# Autodesk Inventor assembly: IFI_FlyWheelAssembly_Jan21
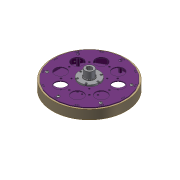
[picture p0: Inventor's stored thumbnail of the model, 180x180]
Saved by Autodesk Inventor 2012 (Build 160160000, 160)
## iProperties
Created: 2012-01-22
Part Number: IFI_FlyWheelAssembly_Jan21
Document SubType Name: Assembly
Designer: JesseK
Mass: 1834.43 g
Surface Area: 3040.14 cm^2
Volume: 862.441 cm^3
Density: 2.12703 g/cm^3
Author: JesseK
## Documents named in this file (3)
- Z:\UserData\Documents\Inventor\team1885frc\Robot2012\Shooter\IFI_FlyWheelAssembly_Jan21.iam
- Z:\UserData\Documents\Inventor\team1885frc\IFI\Imported Components\IFI-WHEEL-ASSY-810-50\IFI-WHEEL-ASSY-810-50.iam
- Z:\UserData\Documents\Inventor\team1885frc\AndyMark\500EX-Key-Hub.ipt
## Components (3 placed, 2 different names)
1. IFI-WHEEL-ASSY-810-50:1 [sub-assembly] — Mate:13, Mate:14, Mate:15, Mate:16, Mate:17, Mate:18
2. 500EX-Key-Hub:1 — Mate:13, Mate:14, Mate:15
3. 500EX-Key-Hub:2 — Mate:16, Mate:17, Mate:18
## Relationships (6: Mate 6)
- Mate:13: IFI-WHEEL-ASSY-810-50:1 ↔ 500EX-Key-Hub:1
- Mate:14: IFI-WHEEL-ASSY-810-50:1 ↔ 500EX-Key-Hub:1
- Mate:15: IFI-WHEEL-ASSY-810-50:1 ↔ 500EX-Key-Hub:1
- Mate:16: IFI-WHEEL-ASSY-810-50:1 ↔ 500EX-Key-Hub:2
- Mate:17: IFI-WHEEL-ASSY-810-50:1 ↔ 500EX-Key-Hub:2
- Mate:18: IFI-WHEEL-ASSY-810-50:1 ↔ 500EX-Key-Hub:2
